# Autodesk Inventor assembly: Assembly
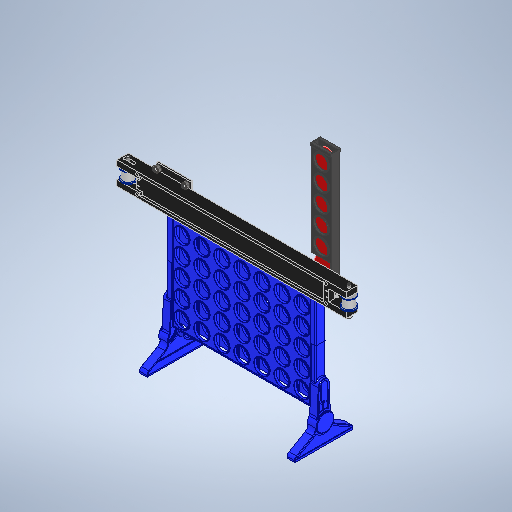
[picture p0: Inventor's stored thumbnail of the model, 512x512]
Saved by Autodesk Inventor 2025.1 (Build 291241020, 241B)
## iProperties
Created: 2024-11-07
Part Number: Assembly
Document SubType Name: Assembly
Designer: leon-
Author: leon-
## Documents named in this file (6)
- C:\Users\leon-\OneDrive\Dokumente\Education\Berkeley\Embedded_Systems\Project\CAD Model\Assembly.iam
- C:\Users\leon-\OneDrive\Dokumente\Education\Berkeley\Embedded_Systems\Project\CAD Model\Connect4_LEG.ipt
- C:\Users\leon-\OneDrive\Dokumente\Education\Berkeley\Embedded_Systems\Project\CAD Model\Connect4_RACK.ipt
- C:\Users\leon-\OneDrive\Dokumente\Education\Berkeley\Embedded_Systems\Project\CAD Model\Sledge.iam
- C:\Users\leon-\OneDrive\Dokumente\Education\Berkeley\Embedded_Systems\Project\CAD Model\Connect4_DISK.ipt
- C:\Users\leon-\OneDrive\Dokumente\Education\Berkeley\Embedded_Systems\Project\CAD Model\Magazine.ipt
## Components (12 placed, 5 different names)
1. Connect4_LEG:1 — Flush:1, Flush:2, Mate:1, Flush:4
2. Connect4_LEG:2 — Mate:2, Mate:3, Flush:3
3. Connect4_RACK:1 — Flush:1, Flush:2, Mate:1, Mate:2, Mate:3, Flush:3, Angle:1, Mate:5, Mate:6, Angle:2, Angle:3, Flush:5, Flush:7
4. Sledge:1 [sub-assembly] — Angle:1, Mate:5, Mate:8, Mate:9, Mate:10, Flush:7
5. Connect4_DISK:1 — Mate:9, Mate:10, Flush:4, Mate:11, Tangent:1
6. Magazine:1 — Mate:11, Tangent:1, Angle:3, Flush:5, Mate:12, Mate:13, Mate:14, Mate:15, Mate:16, Mate:17, Mate:18, Mate:19, Mate:20, Mate:21, Mate:22, Flush:6
7. Connect4_DISK:2 — Mate:18, Mate:19
8. Connect4_DISK:3 — Mate:14, Mate:15
9. Connect4_DISK:4 — Mate:16, Mate:17
10. Connect4_DISK:5 — Mate:20, Mate:21
11. Connect4_DISK:6 — Mate:22, Flush:6
12. Connect4_DISK:7 — Mate:12, Mate:13
## Relationships (32: Mate 21, Flush 7, Angle 3, Tangent 1)
- Flush:1: Connect4_LEG:1 ↔ Connect4_RACK:1
- Flush:2: Connect4_LEG:1 ↔ Connect4_RACK:1
- Mate:1: Connect4_LEG:1 ↔ Connect4_RACK:1
- Mate:2: Connect4_LEG:2 ↔ Connect4_RACK:1
- Mate:3: Connect4_LEG:2 ↔ Connect4_RACK:1
- Flush:3: Connect4_LEG:2 ↔ Connect4_RACK:1
- Angle:1 (0 deg): Connect4_RACK:1 ↔ Sledge:1
- Mate:5: Connect4_RACK:1 ↔ Sledge:1
- Mate:6: Connect4_RACK:1
- Mate:7
- Angle:2 (0 deg): Connect4_RACK:1
- Mate:8: Sledge:1
- Mate:9: Sledge:1 ↔ Connect4_DISK:1
- Mate:10: Sledge:1 ↔ Connect4_DISK:1
- Flush:4: Connect4_LEG:1 ↔ Connect4_DISK:1
- Mate:11: Connect4_DISK:1 ↔ Magazine:1
- Tangent:1: Connect4_DISK:1 ↔ Magazine:1
- Angle:3 (0 deg): Connect4_RACK:1 ↔ Magazine:1
- Flush:5: Connect4_RACK:1 ↔ Magazine:1
- Mate:12: Magazine:1 ↔ Connect4_DISK:7
- Mate:13: Magazine:1 ↔ Connect4_DISK:7
- Mate:14: Magazine:1 ↔ Connect4_DISK:3
- Mate:15: Magazine:1 ↔ Connect4_DISK:3
- Mate:16: Magazine:1 ↔ Connect4_DISK:4
- Mate:17: Magazine:1 ↔ Connect4_DISK:4
- Mate:18: Magazine:1 ↔ Connect4_DISK:2
- Mate:19: Magazine:1 ↔ Connect4_DISK:2
- Mate:20: Magazine:1 ↔ Connect4_DISK:5
- Mate:21: Magazine:1 ↔ Connect4_DISK:5
- Mate:22: Magazine:1 ↔ Connect4_DISK:6
- Flush:6: Magazine:1 ↔ Connect4_DISK:6
- Flush:7 (-53.153 mm): Connect4_RACK:1 ↔ Sledge:1
